# Autodesk Inventor assembly: main_assembly
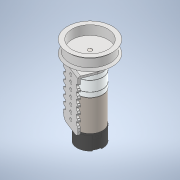
[picture p0: Inventor's stored thumbnail of the model, 180x180]
Saved by Autodesk Inventor 2020 (Build 240168000, 168)
## iProperties
Created: 2020-05-04
Part Number: main_assembly
Document SubType Name: Assembly
Designer: Hesekiel
Author: Hesekiel
## Documents named in this file (4)
- C:\Users\Hesekiel\Documents\Inventor\Uchwyt Aktywny Teleskopu\main_assembly.iam
- C:\Users\Hesekiel\Documents\Inventor\Uchwyt Aktywny Teleskopu\mniejsze_kolo.ipt
- C:\Users\Hesekiel\Documents\Inventor\Uchwyt Aktywny Teleskopu\silnik_full_assembly.iam
- C:\Users\Hesekiel\Documents\Inventor\Uchwyt Aktywny Teleskopu\uchwyt_silnika.ipt
## Components (3 placed, 3 different names)
1. mniejsze_kolo:1 — Insert:1
2. silnik_full_assembly:1 [sub-assembly] — Insert:1, Mate:1, Mate:2, Mate:3
3. uchwyt_silnika:1 — Mate:1, Mate:2, Mate:3
## Relationships (4: Mate 3, Insert 1)
- Insert:1: mniejsze_kolo:1 ↔ silnik_full_assembly:1
- Mate:1: silnik_full_assembly:1 ↔ uchwyt_silnika:1
- Mate:2: silnik_full_assembly:1 ↔ uchwyt_silnika:1
- Mate:3: silnik_full_assembly:1 ↔ uchwyt_silnika:1
